# Autodesk Inventor assembly: machete lineas
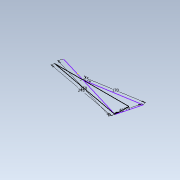
[picture p0: Inventor's stored thumbnail of the model, 180x180]
Saved by Autodesk Inventor 2021 (Build 250183000, 183)
## iProperties
Created: 2021-07-18
Part Number: machete lineas
Document SubType Name: Assembly
Designer: Andrés Holguín
Author: Andrés Holguín
## Documents named in this file (7)
- C:\Users\andre\Downloads\metodos\machete lineas.iam
- C:\Users\andre\Downloads\metodos\Triangulo.ipt
- C:\Users\andre\Downloads\metodos\manivela.ipt
- C:\Users\andre\Downloads\metodos\biela.ipt
- C:\Users\andre\Downloads\metodos\ex.ipt
- C:\Users\andre\Downloads\metodos\rectaImg.ipt
- C:\Users\andre\Downloads\metodos\linea2.ipt
## Components (6 placed, 6 different names)
1. Triangulo:1 — Rotational:1, Slider:1, Rotational:4
2. manivela:1 — Rotational:1, Rotational:2
3. biela:1 — Rotational:2, Rotational:3
4. ex:1 — Slider:1, Rotational:3, Rotational:5
5. rectaImg:1 — Rotational:4, Slider:2
6. linea2:1 — Slider:2, Rotational:5
## Relationships (7: RevoluteJoint 5, TranslationJoint 2)
- Rotational:1 [RevoluteJoint]: Triangulo:1 ↔ manivela:1
- Rotational:2 [RevoluteJoint]: manivela:1 ↔ biela:1
- Slider:1 [TranslationJoint]: Triangulo:1 ↔ ex:1
- Rotational:3 [RevoluteJoint]: biela:1 ↔ ex:1
- Rotational:4 [RevoluteJoint]: Triangulo:1 ↔ rectaImg:1
- Slider:2 [TranslationJoint]: rectaImg:1 ↔ linea2:1
- Rotational:5 [RevoluteJoint]: ex:1 ↔ linea2:1
